# Autodesk Inventor assembly: TMP_Assembly_Ender_Pump
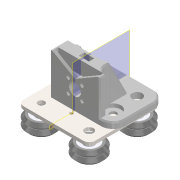
[picture p0: Inventor's stored thumbnail of the model, 180x180]
Saved by Autodesk Inventor 2022 (Build 260153000, 153)
## iProperties
Created: 2021-12-06
Part Number: TMP_Assembly_Ender_Pump
Document SubType Name: Assembly
Designer: diederichbenedict
Author: diederichbenedict
## Documents named in this file (4)
- C:\Users\diederichbenedict\Dropbox\Dokumente\Promotion\PROJECTS\UC2\02_CAD\INVENTOR\uc2_v3\TMP_Assembly_Ender_Pump.iam
- C:\Users\diederichbenedict\Dropbox\Dokumente\Promotion\PROJECTS\UC2\02_CAD\INVENTOR\uc2_v3\00_E Slide Mount v2.ipt
- C:\Users\diederichbenedict\Downloads\00_vslot_slide.ipt
- C:\Users\diederichbenedict\Dropbox\Dokumente\Promotion\PROJECTS\UC2\02_CAD\INVENTOR\uc2_v3\00_Vslot_bearing.ipt
## Components (6 placed, 3 different names)
1. 00_E Slide Mount v2:1 — Passend:1, Passend:2, Passend:3
2. 00_vslot_slide:1 — Einfügen:1, Einfügen:2, Einfügen:3, Einfügen:4, Passend:1, Passend:2, Passend:3
3. 00_Vslot_bearing:1 — Einfügen:1
4. 00_Vslot_bearing:2 — Einfügen:2
5. 00_Vslot_bearing:3 — Einfügen:4
6. 00_Vslot_bearing:4 — Einfügen:3
## Relationships (7: Insert 4, Mate 3)
- Einfügen:1 [Insert] (5 mm): 00_vslot_slide:1 ↔ 00_Vslot_bearing:1
- Einfügen:2 [Insert] (5 mm): 00_vslot_slide:1 ↔ 00_Vslot_bearing:2
- Einfügen:3 [Insert] (5 mm): 00_vslot_slide:1 ↔ 00_Vslot_bearing:4
- Einfügen:4 [Insert] (5 mm): 00_vslot_slide:1 ↔ 00_Vslot_bearing:3
- Passend:1 [Mate]: 00_E Slide Mount v2:1 ↔ 00_vslot_slide:1
- Passend:2 [Mate]: 00_E Slide Mount v2:1 ↔ 00_vslot_slide:1
- Passend:3 [Mate]: 00_E Slide Mount v2:1 ↔ 00_vslot_slide:1
